# Autodesk Inventor assembly: chest_cover
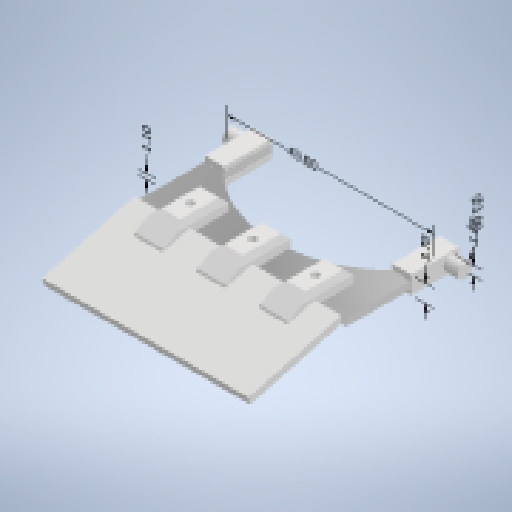
[picture p0: Inventor's stored thumbnail of the model, 512x512]
Saved by Autodesk Inventor 2024.1 (Build 281209000, 209)
## iProperties
Created: 2024-10-12
Part Number: chest_cover
Document SubType Name: Assembly
Designer: hibik
Author: hibik
## Documents named in this file (5)
- C:\Users\hibik\Documents\Robomech\HR\Eglantyne\hard\upper_body\chest\chest_cover.iam
- C:\Users\hibik\Documents\Robomech\HR\Eglantyne\hard\upper_body\chest\chest_cover_base.ipt
- C:\Users\hibik\Documents\Robomech\HR\Eglantyne\hard\upper_body\chest\chest_cover_axis_right.ipt
- C:\Users\hibik\Documents\Robomech\HR\Eglantyne\hard\upper_body\chest\chest_cover_axis_left.ipt
- C:\Users\hibik\Documents\Robomech\HR\Eglantyne\hard\upper_body\chest\chest_cover_cover.ipt
## Components (4 placed, 4 different names)
1. chest_cover_base:1 — メイト:1, フラッシュ:1, メイト:2, フラッシュ:2, メイト:3, メイト:4, 挿入:1, 挿入:2
2. chest_cover_axis_right:1 — メイト:1, フラッシュ:1, メイト:2
3. chest_cover_axis_left:1 — フラッシュ:2, メイト:3, メイト:4
4. chest_cover_cover:1 — 挿入:1, 挿入:2
## Relationships (8: Mate 4, Flush 2, Insert 2)
- メイト:1 [Mate] (0.1 mm): chest_cover_base:1 ↔ chest_cover_axis_right:1
- フラッシュ:1 [Flush]: chest_cover_base:1 ↔ chest_cover_axis_right:1
- メイト:2 [Mate] (0.2 mm): chest_cover_base:1 ↔ chest_cover_axis_right:1
- フラッシュ:2 [Flush]: chest_cover_base:1 ↔ chest_cover_axis_left:1
- メイト:3 [Mate] (0.1 mm): chest_cover_base:1 ↔ chest_cover_axis_left:1
- メイト:4 [Mate] (0.2 mm): chest_cover_base:1 ↔ chest_cover_axis_left:1
- 挿入:1 [Insert]: chest_cover_base:1 ↔ chest_cover_cover:1
- 挿入:2 [Insert]: chest_cover_base:1 ↔ chest_cover_cover:1
